# Autodesk Inventor assembly: WheelIntake4.0
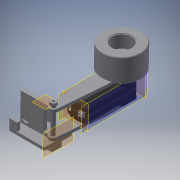
[picture p0: Inventor's stored thumbnail of the model, 180x180]
Saved by Autodesk Inventor 2017 (Build 210142000, 142)
## iProperties
Created: 2017-12-13
Part Number: WheelIntake4.0
Document SubType Name: Assembly
Designer: User
Author: User
## Documents named in this file (6)
- C:\Robotics\CAD\2017-18_CAD\WheelIntake5.0.iam
- C:\Robotics\CAD\COTSParts\Rev\REV-41-1300.ipt
- C:\Robotics\CAD\COTSParts\Fasteners\97345A171_TYPE 316 STAINLESS STEEL SHOULDER SCREW.ipt
- C:\Robotics\CAD\COTSParts\Wheels\2.5inFoamWheel250TMD.ipt
- C:\Robotics\CAD\2017-18_CAD\WheelIntake5.0Base.ipt
- C:\Robotics\CAD\2017-18_CAD\WheelIntake5.0Mount.ipt
## Components (5 placed, 5 different names)
1. REV-41-1300:1 — Insert:2, Insert:3
2. 97345A171_TYPE 316 STAINLESS STEEL SHOULDER SCREW:1 — Insert:1, Insert:5, Insert:6
3. 2.5inFoamWheel250TMD:1 — Mate:1, Insert:4
4. WheelIntake5.0Base:1 — Mate:1, Insert:5, Insert:6
5. WheelIntake5.0Mount:1 — Insert:1, Insert:2, Insert:3, Insert:4
## Relationships (7: Insert 6, Mate 1)
- Mate:1 (5.4864 mm): 2.5inFoamWheel250TMD:1 ↔ WheelIntake5.0Base:1
- Insert:1: 97345A171_TYPE 316 STAINLESS STEEL SHOULDER SCREW:1 ↔ WheelIntake5.0Mount:1
- Insert:2: REV-41-1300:1 ↔ WheelIntake5.0Mount:1
- Insert:3: REV-41-1300:1 ↔ WheelIntake5.0Mount:1
- Insert:4: 2.5inFoamWheel250TMD:1 ↔ WheelIntake5.0Mount:1
- Insert:5: 97345A171_TYPE 316 STAINLESS STEEL SHOULDER SCREW:1 ↔ WheelIntake5.0Base:1
- Insert:6: 97345A171_TYPE 316 STAINLESS STEEL SHOULDER SCREW:1 ↔ WheelIntake5.0Base:1
